# Autodesk Inventor assembly: Arm for Gen 2
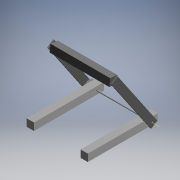
[picture p0: Inventor's stored thumbnail of the model, 180x180]
Saved by Autodesk Inventor 2019 (Build 230136000, 136)
## iProperties
Part Number: Arm for Gen 2
Document SubType Name: Assembly
Designer: Delta
Author: Delta
## Documents named in this file (6)
- C:\Robotics\2019-20_CAD\Collection\Arm for Gen 2.iam
- C:\Robotics\2019-20_CAD\Collection\30x30 pillars.ipt
- C:\Robotics\2019-20_CAD\Collection\12 Inch Hex Axle.ipt
- C:\Robotics\COTSParts\Sprockets - AndyMark\615106.ipt
- C:\Robotics\2019-20_CAD\Collection\bar arms.ipt
- C:\Robotics\2019-20_CAD\Collection\Claw holding bars.ipt
## Components (7 placed, 5 different names)
1. 30x30 pillars:1 — Mate:2, Flush:2, Mate:7, Mate:11
2. 30x30 pillars:2 — Mate:3, Flush:2, Mate:11, Mate:12
3. 12 Inch Hex Axle:1 — Mate:2, Mate:3, Mate:5, Mate:6, Flush:4, Mate:8
4. 615106:1 — Mate:5, Mate:12, Mate:13
5. bar arms:1 — Mate:6, Mate:7, Flush:4, Flush:5
6. bar arms:2 — Mate:8, Flush:5, Mate:13, Mate:14, Mate:15
7. Claw holding bars:1 — Mate:14, Mate:15
## Relationships (14: Mate 11, Flush 3)
- Mate:2: 30x30 pillars:1 ↔ 12 Inch Hex Axle:1
- Mate:3: 30x30 pillars:2 ↔ 12 Inch Hex Axle:1
- Flush:2: 30x30 pillars:1 ↔ 30x30 pillars:2
- Mate:5: 12 Inch Hex Axle:1 ↔ 615106:1
- Mate:6: 12 Inch Hex Axle:1 ↔ bar arms:1
- Mate:7: 30x30 pillars:1 ↔ bar arms:1
- Flush:4: 12 Inch Hex Axle:1 ↔ bar arms:1
- Mate:8: 12 Inch Hex Axle:1 ↔ bar arms:2
- Flush:5: bar arms:1 ↔ bar arms:2
- Mate:11 (203.2 mm): 30x30 pillars:1 ↔ 30x30 pillars:2
- Mate:12: 30x30 pillars:2 ↔ 615106:1
- Mate:13: 615106:1 ↔ bar arms:2
- Mate:14: bar arms:2 ↔ Claw holding bars:1
- Mate:15: bar arms:2 ↔ Claw holding bars:1
